# Autodesk Inventor assembly: top_3
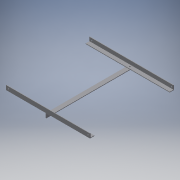
[picture p0: Inventor's stored thumbnail of the model, 180x180]
Saved by Autodesk Inventor 2017 (Build 210142000, 142)
## iProperties
Created: 2018-10-24
Part Number: top_3
Document SubType Name: Assembly
Designer: ddeboer
Author: ddeboer
## Documents named in this file (3)
- C:\Users\ddeboer\Desktop\snap_holder\top_3.iam
- C:\Users\ddeboer\Desktop\snap_holder\angle_L1.ipt
- C:\Users\ddeboer\Desktop\snap_holder\angle_L104.ipt
## Components (3 placed, 2 different names)
1. angle_L1:1 — Insert:1, Insert:2, Flush:1, Flush:2
2. angle_L104:1 — Insert:2, Flush:2
3. angle_L104:2 — Insert:1, Flush:1
## Relationships (4: Insert 2, Flush 2)
- Insert:1: angle_L1:1 ↔ angle_L104:2
- Insert:2: angle_L1:1 ↔ angle_L104:1
- Flush:1: angle_L1:1 ↔ angle_L104:2
- Flush:2: angle_L1:1 ↔ angle_L104:1
